# Autodesk Inventor assembly: DetektorElektronik_Stage2
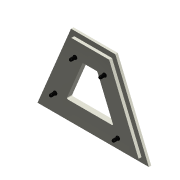
[picture p0: Inventor's stored thumbnail of the model, 180x180]
Saved by Autodesk Inventor 2018.2 (Build 222227000, 227)
## iProperties
Company: Fraunhofer ILT
Created: 2018-11-09
Part Number: DetektorElektronik_Stage2
Material: geeigneten Werkstoff auswählen !
Document SubType Name: Assembly
Designer: N.Grubert
Title: =Description
Author: N.Grubert
## Documents named in this file (3)
- V:\A340\2018\DOKUMENTATION\COSIMA\COSIMA-Laserstar\CAD\Detektormodul\DetektorElektronik_Stage2.iam
- V:\A340\2018\DOKUMENTATION\COSIMA\COSIMA-Laserstar\CAD\Detektormodul\Stage2.ipt
- V:\A340\2018\DOKUMENTATION\COSIMA\COSIMA-Laserstar\CAD\Detektormodul\Photodiodendummie.ipt
## Components (5 placed, 2 different names)
1. Stage2:1 — Passend:1, Passend:2, Passend:3, Passend:4, Passend:5, Passend:6, Passend:7
2. Photodiodendummie:1 — Passend:7
3. Photodiodendummie:2 — Passend:6
4. Photodiodendummie:3 — Passend:5
5. Photodiodendummie:4 — Passend:4
## Relationships (7: Mate 7)
- Passend:1 [Mate]: Stage2:1
- Passend:2 [Mate]: Stage2:1
- Passend:3 [Mate]: Stage2:1
- Passend:4 [Mate]: Stage2:1 ↔ Photodiodendummie:4
- Passend:5 [Mate]: Stage2:1 ↔ Photodiodendummie:3
- Passend:6 [Mate]: Stage2:1 ↔ Photodiodendummie:2
- Passend:7 [Mate]: Stage2:1 ↔ Photodiodendummie:1
